# Autodesk Inventor assembly: RobotArm
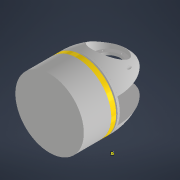
[picture p0: Inventor's stored thumbnail of the model, 180x180]
Saved by Autodesk Inventor 2021 (Build 250183000, 183)
## iProperties
Created: 2022-10-01
Part Number: RobotArm
Document SubType Name: Assembly
Designer: MicnedSQ
Author: MicnedSQ
## Documents named in this file (3)
- C:\Users\MicnedSQ\Desktop\V1\RobotArm.iam
- C:\Users\MicnedSQ\Desktop\V1\Base\Base.iam
- C:\Users\MicnedSQ\Desktop\V1\RotatingBase\RotatingBase.iam
## Components (2 placed, 2 different names)
1. Base:1 [sub-assembly] — Obrotowe:1
2. RotatingBase:1 [sub-assembly] — Obrotowe:1
## Relationships (1: RevoluteJoint 1)
- Obrotowe:1 [RevoluteJoint]: Base:1 ↔ RotatingBase:1
